# Autodesk Inventor assembly: Assembly suelo
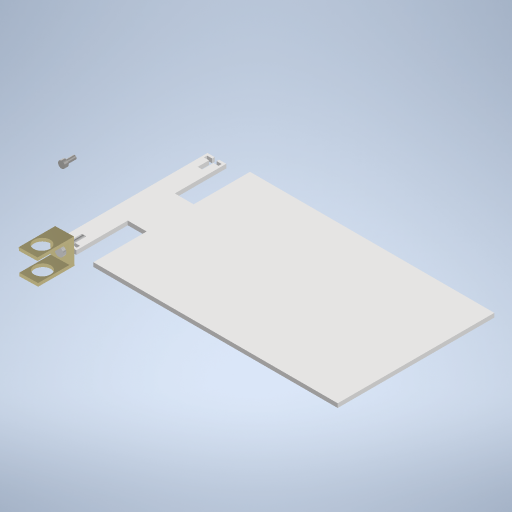
[picture p0: Inventor's stored thumbnail of the model, 512x512]
Saved by Autodesk Inventor 2024 (Build 280153000, 153)
## iProperties
Created: 2023-05-06
Part Number: Assembly suelo
Document SubType Name: Assembly
Designer: Diego
Author: Diego
## Documents named in this file (5)
- C:\Users\Diego\Desktop\Proyecto2_micros\Assembly suelo.iam
- C:\Users\Diego\Desktop\Proyecto2_micros\suelo_imp.ipt
- C:\Users\Diego\Desktop\Proyecto2_micros\tornillo_5_5_10_5.ipt
- C:\Users\Diego\Desktop\Proyecto2_micros\llanta_1.ipt
- C:\Users\Diego\Desktop\Proyecto2_micros\tornillo_7_21.ipt
## Components (4 placed, 4 different names)
1. suelo_imp:1 — Rigid:3, Rotational:1
2. tornillo_5_5_10_5:1
3. llanta_1:1 — Rotational:1
4. tornillo_7_21:1 — Rigid:3
## Relationships (2: WeldJoint 1, RevoluteJoint 1)
- Rigid:3 [WeldJoint]: suelo_imp:1 ↔ tornillo_7_21:1
- Rotational:1 [RevoluteJoint]: suelo_imp:1 ↔ llanta_1:1
